# Autodesk Inventor assembly: lifting pulley assembled
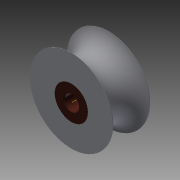
[picture p0: Inventor's stored thumbnail of the model, 180x180]
Saved by Autodesk Inventor 2015 (Build 190159000, 159)
## iProperties
Created: 2014-10-25
Part Number: lifting pulley assembled
Document SubType Name: Assembly
Designer: jesse
Author: jesse
## Documents named in this file (3)
- C:\Users\jesse\Desktop\robot\lift\lifting pulley assembled.iam
- C:\Users\jesse\Desktop\robot\stock parts\bronze_bushing_2012\bronze_bushing_2012.ipt
- C:\Users\jesse\Desktop\robot\lift\lifting pulley.ipt
## Components (2 placed, 2 different names)
1. bronze_bushing_2012:1 — Mate:1, Mate:2
2. lifting pulley:1 — Mate:1, Mate:2
## Relationships (2: Mate 2)
- Mate:1: bronze_bushing_2012:1 ↔ lifting pulley:1
- Mate:2: bronze_bushing_2012:1 ↔ lifting pulley:1
